# Autodesk Inventor assembly: FinalAssembly
(part 3 of 3)
- Flush:502 (1.905 mm): ServoWithShaftAssembly:1 ↔ HallEffectSpoolSensorMount2:1
- Mate:1110: NarrowHexNutThread_5_40:210 ↔ HallEffectSpoolSensorMount2:1
- Angle:80 (-20 deg): ServoWithShaftAssembly:1 ↔ HallEffectSpoolSensorMount2:1
- Mate:1111: HallEffectSpoolSensorMount2:1 ↔ HallEffectSensor:1
- Flush:503: HallEffectSpoolSensorMount2:1 ↔ HallEffectSensor:1
- Mate:1112: HallEffectSpoolSensorMount2:1 ↔ HallEffectSensor:1
- Mate:1113: HallEffectSpoolSensorMount2:1 ↔ aftServoSectionThreadedRodThread_5_40:2
- Flush:504: largeIdlerPinion:4 ↔ smallIdlerPinion:7
- Mate:1114 (6.096 mm): frontServoAttachmentPlate:1 ↔ largeIdlerPinion:4
- Flush:505 (2.54 mm): CarriageConnectorShaft:1 ↔ smallIdlerPinion:8
- Mate:1115: largeIdlerPinion:4 ↔ SpoolCarrageMagnetMountREV2:1
- Mate:1116: largeIdlerPinion:4 ↔ SpoolCarrageMagnetMountREV2:1
- Mate:1117: SpoolCarrageMagnetMountREV2:1 ↔ EncoderMagnet:3
- Mate:1118: SpoolCarrageMagnetMountREV2:1 ↔ EncoderMagnet:3
- Mate:1120: HallEffectSpoolSensorMount3Brace:1 ↔ aftServoSectionThreadedRodThread_5_40:6
- Mate:1121: HallEffectSpoolSensorMount3Brace:1 ↔ aftServoSectionThreadedRodThread_5_40:5
- Mate:1122: HallEffectSpoolSensorMount3:1 ↔ HallEffectSpoolSensorMount3Brace:1
- Mate:1123: HallEffectSpoolSensorMount3:1 ↔ HallEffectSpoolSensorMount3Brace:1
- Mate:1124: NarrowHexNutThread_5_40:211 ↔ aftServoSectionThreadedRodThread_5_40:5
- Mate:1125: HallEffectSpoolSensorMount3Brace:1 ↔ NarrowHexNutThread_5_40:211
- Mate:1126: NarrowHexNutThread_5_40:212 ↔ aftServoSectionThreadedRodThread_5_40:5
- Mate:1127: HallEffectSpoolSensorMount3Brace:1 ↔ NarrowHexNutThread_5_40:212
- Angle:81 (0 deg): NarrowHexNutThread_5_40:211 ↔ NarrowHexNutThread_5_40:212
- Angle:82 (0 deg): HitecServoAssembly:1 ↔ NarrowHexNutThread_5_40:211
- Mate:1128 (12.7 mm): frontServoAttachmentPlate:1 ↔ HallEffectSpoolSensorMount3Brace:1
- Mate:1129: HallEffectSpoolSensorMount3Brace:1 ↔ Bolt_ButtonHead_Hex_Thread_M3_10mm:4
- Mate:1130: HallEffectSpoolSensorMount3:1 ↔ Bolt_ButtonHead_Hex_Thread_M3_10mm:4
- Angle:83 (0 deg): HallEffectSpoolSensorMount3:1 ↔ Bolt_ButtonHead_Hex_Thread_M3_10mm:4
- Mate:1131: Bolt_ButtonHead_Hex_Thread_M3_10mm:4 ↔ HexNutThread_M3:6
- Mate:1132: HallEffectSpoolSensorMount3Brace:1 ↔ HexNutThread_M3:6
- Angle:84 (0 deg): HitecServoAssembly:2 ↔ HexNutThread_M3:6
- Mate:1133: HallEffectSpoolSensorMount3:1 ↔ HallEffectSensor:2
- Mate:1134: HallEffectSpoolSensorMount3:1 ↔ HallEffectSensor:2
- Flush:506: HallEffectSpoolSensorMount3:1 ↔ HallEffectSensor:2
- Angle:85 (0 deg): pistonSealingWallRear:1
- Angle:86 (0 deg): pistonSealingWallFront:1
- Mate:1135: ThrustBearingMount:1 ↔ HallEffectSpoolSensorMount3:2
- Mate:1136: ThrustBearingMount:1 ↔ HallEffectSpoolSensorMount3:2
- Mate:1137: HallEffectSpoolSensorMount3:2 ↔ ScrewPlastic_4_20_.5inch:38
- Mate:1138: HallEffectSpoolSensorMount3:2 ↔ ScrewPlastic_4_20_.5inch:38
- Angle:87 (0 deg): limitSwitchHolder2:1 ↔ HallEffectSpoolSensorMount3:2
- Mate:1139: NarrowHexNutThread_5_40:213 ↔ midshipsThreadedRodThread_5_40:6
- Mate:1140: ArduinoNanoHolder:1 ↔ NarrowHexNutThread_5_40:213
- Angle:88 (0 deg): ArduinoNanoHolder:1 ↔ NarrowHexNutThread_5_40:213
- Mate:1141: NarrowHexNutThread_5_40:214 ↔ midshipsThreadedRodThread_5_40:1
- Mate:1142: ArduinoNanoHolder:1 ↔ NarrowHexNutThread_5_40:214
- Angle:89 (0 deg): ArduinoNanoHolder:1 ↔ NarrowHexNutThread_5_40:214
- Mate:1143: RelayHolderREV2:1 ↔ midshipsThreadedRodThread_5_40:1
- Mate:1144: RelayHolderREV2:1 ↔ midshipsThreadedRodThread_5_40:6
- Mate:1145: RelayHolderREV2:1 ↔ RelayModule:1
- Mate:1146: RelayHolderREV2:1 ↔ RelayModule:1
- Angle:90 (0 deg): RelayHolderREV2:1 ↔ RelayModule:1
- Mate:1147: FixedCylinderWireStorage:1 ↔ SlipRingAssy:1
- Mate:1148 (9.525 mm): SpoolSectionSealingWallFront:1 ↔ SlipRingAssy:1
- Mate:1149: midshipsThreadedRodThread_5_40:3 ↔ batteryHolderBracket:2
- Mate:1150: midshipsThreadedRodThread_5_40:4 ↔ batteryHolderBracket:2
- Mate:1151 (127 mm): forwardBallastSealingWallFront:1 ↔ batteryHolderBracket:2
- Mate:1152: DriveBattery:2 ↔ batteryHolderBracket:2
- Mate:1153: DriveBattery:2 ↔ batteryHolderBracket:3
- Mate:1154 (25.4 mm): foreElectronicsSealingWallRear:1 ↔ DriveBattery:2
- Mate:1155: midshipsThreadedRodThread_5_40:4 ↔ NarrowHexNutThread_5_40:215
- Mate:1156: batteryHolderBracket:2 ↔ NarrowHexNutThread_5_40:215
- Angle:91 (0 deg): batteryHolderBracket:2 ↔ NarrowHexNutThread_5_40:215
- Mate:1157: midshipsThreadedRodThread_5_40:4 ↔ NarrowHexNutThread_5_40:216
- Mate:1158: batteryHolderBracket:2 ↔ NarrowHexNutThread_5_40:216
- Angle:92 (0 deg): batteryHolderBracket:2 ↔ NarrowHexNutThread_5_40:216
- Mate:1159: midshipsThreadedRodThread_5_40:3 ↔ NarrowHexNutThread_5_40:217
- Mate:1160: batteryHolderBracket:2 ↔ NarrowHexNutThread_5_40:217
- Angle:93 (0 deg): batteryHolderBracket:2 ↔ NarrowHexNutThread_5_40:217
- Mate:1161: midshipsThreadedRodThread_5_40:3 ↔ NarrowHexNutThread_5_40:218
- Mate:1162: batteryHolderBracket:2 ↔ NarrowHexNutThread_5_40:218
- Angle:94 (0 deg): batteryHolderBracket:2 ↔ NarrowHexNutThread_5_40:218
- Mate:1163: foreElectronicsSealingWallRear:1 ↔ PreloadSpacerForThreadedRods:1
- Mate:1164: PreloadSpacerForThreadedRods:1 ↔ midshipsThreadedRodThread_5_40:4
- Mate:1165: PreloadSpacerForThreadedRods:1 ↔ NarrowHexNutThread_5_40:167
- Mate:1166: midshipsThreadedRodThread_5_40:2 ↔ NarrowHexNutThread_5_40:227
- Mate:1167: PreloadSpacerForThreadedRods:1 ↔ NarrowHexNutThread_5_40:227
- Angle:95 (0 deg): NarrowHexNutThread_5_40:166 ↔ NarrowHexNutThread_5_40:227
- Mate:1168: midshipsThreadedRodThread_5_40:6 ↔ NarrowHexNutThread_5_40:233
- Mate:1169: PreloadSpacerForThreadedRods:1 ↔ NarrowHexNutThread_5_40:233
- Angle:96 (0 deg): NarrowHexNutThread_5_40:231 ↔ NarrowHexNutThread_5_40:233
- Mate:1170 (6.35 mm): RelayHolderREV2:1 ↔ NarrowHexNutThread_5_40:161
- Mate:1171: midshipsThreadedRodThread_5_40:6 ↔ NarrowHexNutThread_5_40:236
- Mate:1172: RelayHolderREV2:1 ↔ NarrowHexNutThread_5_40:236
- Angle:97 (0 deg): RelayHolderREV2:1 ↔ NarrowHexNutThread_5_40:236
- Mate:1173: midshipsThreadedRodThread_5_40:6 ↔ NarrowHexNutThread_5_40:239
- Mate:1174: midshipsThreadedRodThread_5_40:1 ↔ NarrowHexNutThread_5_40:238
- Mate:1175: midshipsThreadedRodThread_5_40:1 ↔ NarrowHexNutThread_5_40:237
- Mate:1176: RelayHolderREV2:1 ↔ NarrowHexNutThread_5_40:237
- Angle:98 (0 deg): NarrowHexNutThread_5_40:161 ↔ NarrowHexNutThread_5_40:237
- Mate:1177: RelayHolderREV2:1 ↔ NarrowHexNutThread_5_40:238
- Angle:99 (0 deg): NarrowHexNutThread_5_40:237 ↔ NarrowHexNutThread_5_40:238
- Mate:1178: RelayHolderREV2:1 ↔ NarrowHexNutThread_5_40:239
- Angle:100 (0 deg): NarrowHexNutThread_5_40:236 ↔ NarrowHexNutThread_5_40:239
- Mate:1179: aftSectionAirtightCap:2 ↔ aftMount:1
- Angle:101 (0 deg): ASDSAssembly:1 ↔ aftMount:1
- Flush:507 (38.1 mm): aftSectionAirtightCap:2 ↔ aftMount:1
- Angle:102 (0 deg): HitecServoAssembly:1 ↔ ASDSAssembly:1
- Mate:1180: ASDSAssembly:1 ↔ aftMount:1
- Flush:508 (26.67 mm): aftSectionAirtightCap:2 ↔ ASDSAssembly:1
- Flush:509 (206.375 mm): aftSectionAirtightCap:2 ↔ ASDSAttachmentAssemblyUpdated:1
## Named parameters: d30_d28 = 0 mm, d31_d29 = 0 mm
